# Autodesk Inventor assembly: 0005-00-03 Y axis
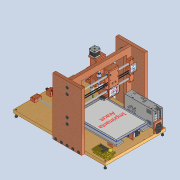
[picture p0: Inventor's stored thumbnail of the model, 180x180]
Saved by Autodesk Inventor 2020 (Build 240168000, 168)
## iProperties
Created: 2020-12-18
Part Number: 0005-00-03 Y axis
Document SubType Name: Assembly
Designer: Iulian Bors
Mass: 17144.8 g
Surface Area: 27601.7 cm^2
Volume: 16303.9 cm^3
Density: 1.05157 g/cm^3
Author: Iulian Bors
## iProperties of the stored document Part 1.ipt
Created: 2020-12-18
Part Number: Part 1
Material: Generic
Document SubType Name: Modeling
Designer: Iulian Bors
Density: 1 g/cm^3
Appearance: Default
Mass: 0.27605 g
Surface Area: 6.48852 cm^2
Volume: 0.27605 cm^3
Author: Iulian Bors
Revision Number: NONE
## iProperties of the stored document Part 2.ipt
Created: 2020-12-18
Part Number: Part 2
Material: Generic
Document SubType Name: Modeling
Designer: Iulian Bors
Density: 1 g/cm^3
Appearance: Default
Mass: 0.0253291 g
Surface Area: 2.0565 cm^2
Volume: 0.0253291 cm^3
Author: Iulian Bors
Revision Number: NONE
## iProperties of the stored document Needle.iam
Created: 2020-01-23
Part Number: Needle
Document SubType Name: Assembly
Designer: Iulian Bors
Mass: 0.301379 g
Surface Area: 8.54503 cm^2
Volume: 0.301379 cm^3
Density: 1 g/cm^3
Title: /vol/tmp/translate-4006329005178005204/5e293bbb2de6b7156cc2e2d4.step
## Documents named in this file (60)
- Z:\I.A.B\Proiecte\0005 I.A.B 3d 2.0 Imprimanta aracet\10 Mecanic\0005-00-03 Y axis.iam
- Z:\I.A.B\Proiecte\0005 I.A.B 3d 2.0 Imprimanta aracet\10 Mecanic\0005-10-001-Batiu.ipt
- Z:\I.A.B\Proiecte\0005 I.A.B 3d 2.0 Imprimanta aracet\20 Electric\0005-20-01 Assembly Arduino Mega RAMPS 1.4.iam
- Z:\I.A.B\Proiecte\0005 I.A.B 3d 2.0 Imprimanta aracet\10 Mecanic\Foaie A4.ipt
- Z:\I.A.B\Proiecte\0005 I.A.B 3d 2.0 Imprimanta aracet\10 Mecanic\Seringa\body 20ml_Défaut.ipt
- Z:\I.A.B\Proiecte\0005 I.A.B 3d 2.0 Imprimanta aracet\10 Mecanic\Seringa\Plunger Assembly_Défaut.iam
- **Z:\I.A.B\Proiecte\0005 I.A.B 3d 2.0 Imprimanta aracet\10 Mecanic\0005-00-03 Y axis.iam*LocalDocs*xAaaaqeaaAaaaaaaaAaaaq3zaLd*Needle.iam
- Z:\I.A.B\Proiecte\0005 I.A.B 3d 2.0 Imprimanta aracet\10 Mecanic\0005-10-003 Actionare seringa.ipt
- Z:\I.A.B\Proiecte\0005 I.A.B 3d 2.0 Imprimanta aracet\10 Mecanic\0005-10-004 Actionare 2 seringa.ipt
- Z:\I.A.B\Proiecte\0005 I.A.B 3d 2.0 Imprimanta aracet\10 Mecanic\0005-10-1004 Piulita.ipt
- Z:\I.A.B\Proiecte\0005 I.A.B 3d 2.0 Imprimanta aracet\10 Mecanic\0005-10-10-1003 LeadScrew 8mm x 2mmPitch.ipt
- Z:\I.A.B\Proiecte\0005 I.A.B 3d 2.0 Imprimanta aracet\10 Mecanic\0005-10-1005 ISO 1224-1 - 10 - 8 x 22 x 7.ipt
- Z:\I.A.B\Proiecte\0005 I.A.B 3d 2.0 Imprimanta aracet\10 Mecanic\0005-10-005.ipt
- Z:\I.A.B\Proiecte\0005 I.A.B 3d 2.0 Imprimanta aracet\10 Mecanic\0005-10-006 Capac rulment.ipt
- Z:\I.A.B\Proiecte\0005 I.A.B 3d 2.0 Imprimanta aracet\10 Mecanic\0005-10-1002  Hub.ipt
- Z:\I.A.B\Proiecte\0005 I.A.B 3d 2.0 Imprimanta aracet\10 Mecanic\0005-10-1001 NEMA17 - Motor de passo.ipt
- Z:\I.A.B\Proiecte\0005 I.A.B 3d 2.0 Imprimanta aracet\10 Mecanic\0005-10-007Suport nema.ipt
- Z:\I.A.B\Proiecte\0005 I.A.B 3d 2.0 Imprimanta aracet\10 Mecanic\0005-10-008.ipt
- Z:\I.A.B\Proiecte\0005 I.A.B 3d 2.0 Imprimanta aracet\10 Mecanic\0005-10-009.ipt
- Z:\I.A.B\Proiecte\0005 I.A.B 3d 2.0 Imprimanta aracet\10 Mecanic\0005-10-010.ipt
- Z:\I.A.B\Proiecte\0005 I.A.B 3d 2.0 Imprimanta aracet\10 Mecanic\0005-10-1006 Bara rectificata.ipt
- Z:\I.A.B\Proiecte\0005 I.A.B 3d 2.0 Imprimanta aracet\10 Mecanic\0005-10-011.ipt
- Z:\I.A.B\Proiecte\0005 I.A.B 3d 2.0 Imprimanta aracet\10 Mecanic\0005-10-012.ipt
- Z:\I.A.B\Proiecte\0005 I.A.B 3d 2.0 Imprimanta aracet\10 Mecanic\0005-10-1007 Bara rectificata.ipt
- Z:\I.A.B\Proiecte\0005 I.A.B 3d 2.0 Imprimanta aracet\10 Mecanic\0005-10-013 Bed.ipt
- Z:\I.A.B\Proiecte\0005 I.A.B 3d 2.0 Imprimanta aracet\10 Mecanic\0005-10-1008 Bara rectificata.ipt
- Z:\I.A.B\Proiecte\0005 I.A.B 3d 2.0 Imprimanta aracet\10 Mecanic\0005-10-014 Suport Bed.ipt
- Z:\I.A.B\Proiecte\0005 I.A.B 3d 2.0 Imprimanta aracet\10 Mecanic\0005-10-1009 LM10uu.ipt
- Z:\I.A.B\Proiecte\0005 I.A.B 3d 2.0 Imprimanta aracet\10 Mecanic\0005-10-002 Suport1 Seringa.ipt
- Z:\I.A.B\Proiecte\0005 I.A.B 3d 2.0 Imprimanta aracet\10 Mecanic\0005-10-016.ipt
- Z:\I.A.B\Proiecte\0005 I.A.B 3d 2.0 Imprimanta aracet\10 Mecanic\0005-10-015 suport tija.ipt
- Z:\I.A.B\Proiecte\0005 I.A.B 3d 2.0 Imprimanta aracet\10 Mecanic\0005-10-017 Batiu 2.ipt
- Z:\I.A.B\Proiecte\0005 I.A.B 3d 2.0 Imprimanta aracet\10 Mecanic\0005-10-1010 GT2 Timing Pulley 20 Tooth.ipt
- Z:\I.A.B\Proiecte\0005 I.A.B 3d 2.0 Imprimanta aracet\10 Mecanic\0005-10-1011 16T W6 B3 Without T_Shrinkwrap_1.ipt
- Z:\I.A.B\Proiecte\0005 I.A.B 3d 2.0 Imprimanta aracet\10 Mecanic\Surub M4 saiba piulita.iam
- Z:\I.A.B\Proiecte\0005 I.A.B 3d 2.0 Imprimanta aracet\10 Mecanic\0005-10-018 intinzator x.ipt
- Z:\I.A.B\Proiecte\0005 I.A.B 3d 2.0 Imprimanta aracet\10 Mecanic\0005-10-1015 curea x.ipt
- Z:\I.A.B\Proiecte\0005 I.A.B 3d 2.0 Imprimanta aracet\10 Mecanic\0005-10-019 intinzator y.ipt
- Z:\I.A.B\Proiecte\0005 I.A.B 3d 2.0 Imprimanta aracet\10 Mecanic\0005-10-1016 curea Y.ipt
- Z:\I.A.B\Proiecte\0005 I.A.B 3d 2.0 Imprimanta aracet\20 Electric\0005-20-1003 Switch.ipt
- Z:\I.A.B\Proiecte\0005 I.A.B 3d 2.0 Imprimanta aracet\10 Mecanic\0005-10-021 suport senzor z.ipt
- Z:\I.A.B\Proiecte\0005 I.A.B 3d 2.0 Imprimanta aracet\10 Mecanic\0005-10-020 suport motor y.ipt
- Z:\I.A.B\Proiecte\0005 I.A.B 3d 2.0 Imprimanta aracet\10 Mecanic\0005-10-023 Suport motor x.ipt
- Z:\I.A.B\Proiecte\0005 I.A.B 3d 2.0 Imprimanta aracet\10 Mecanic\0005-10-024.ipt
- Z:\I.A.B\Proiecte\0005 I.A.B 3d 2.0 Imprimanta aracet\10 Mecanic\0005-10-1000 LM8.ipt
- Z:\I.A.B\Proiecte\0005 I.A.B 3d 2.0 Imprimanta aracet\10 Mecanic\0005-10-1018 tija 8.ipt
- Z:\I.A.B\Proiecte\0005 I.A.B 3d 2.0 Imprimanta aracet\10 Mecanic\Surub M3 40 mm.iam
- Z:\I.A.B\Proiecte\0005 I.A.B 3d 2.0 Imprimanta aracet\10 Mecanic\0005-10-025 Activator senzor Y.ipt
- Z:\I.A.B\Proiecte\0005 I.A.B 3d 2.0 Imprimanta aracet\10 Mecanic\0005-10-1022 tiping screw.ipt
- Z:\I.A.B\Proiecte\0005 I.A.B 3d 2.0 Imprimanta aracet\10 Mecanic\0005-10-1023 ISO 4018 - M8 x 40.ipt
- Z:\I.A.B\Proiecte\0005 I.A.B 3d 2.0 Imprimanta aracet\10 Mecanic\0005-10-026 Suport DC in.ipt
- Z:\I.A.B\Proiecte\0005 I.A.B 3d 2.0 Imprimanta aracet\20 Electric\00005-20-1004 PowerSupplyLedMax500.ipt
- Z:\I.A.B\Proiecte\0005 I.A.B 3d 2.0 Imprimanta aracet\20 Electric\005-20-1004.ipt
- Z:\I.A.B\Proiecte\0005 I.A.B 3d 2.0 Imprimanta aracet\10 Mecanic\0005-10-027 suport nema Z.ipt
- Z:\I.A.B\Proiecte\0005 I.A.B 3d 2.0 Imprimanta aracet\10 Mecanic\0005-10-1025 ISO 4762 - M3 x 16ISO.ipt
- Z:\I.A.B\Proiecte\0005 I.A.B 3d 2.0 Imprimanta aracet\10 Mecanic\0005-10-1020 ISO 7089 - 3 - 140 HV(1).ipt
- **Z:\I.A.B\Proiecte\0005 I.A.B 3d 2.0 Imprimanta aracet\0005-00-00 Ansamblu_General.iam*LocalDocs*xAaaaaecaAaaaaaaaAaaaqfy1Od*Part 1.ipt
- **Z:\I.A.B\Proiecte\0005 I.A.B 3d 2.0 Imprimanta aracet\0005-00-00 Ansamblu_General.iam*LocalDocs*xAaaaa4baAaaaaaaaAaaaq4bsZa*Part 2.ipt
- **Z:\I.A.B\Proiecte\0005 I.A.B 3d 2.0 Imprimanta aracet\0005-00-00 Ansamblu_General.iam*LocalDocs*xAaaaqeaaAaaaaaaaAaaaq3zaLd*Needle.iam
- Z:\I.A.B\Proiecte\0005 I.A.B 3d 2.0 Imprimanta aracet\10 Mecanic\Seringa\21-gauge-needle-1.snapshot.2\Needle.step
## Components (116 placed, 54 different names)
1. 0005-10-001-Batiu.ipt:1 — Mate:3, Angle:1, Mate:43, Angle:7, Angle:8, Angle:10, Mate:62, Flush:36, Mate:64, Flush:38, Mate:109, Mate:90, Mate:91, Mate:92, Mate:93, Mate:101, Mate:108, Flush:60, Mate:116, Insert:32, Insert:33, Mate:127, Mate:131, Mate:143, Mate:147, Flush:73, Insert:41, Insert:42
2. 0005-20-01 Assembly Arduino Mega RAMPS 1.4.iam:2 [sub-assembly] — Mate:147, Flush:73
3. Foaie A4.ipt:3 — Mate:3, Angle:1, Flush:29, Flush:30, Mate:47
4. Needle.iam:4 [sub-assembly] — Insert:14
5. 0005-10-10-1003 LeadScrew 8mm x 2mmPitch.ipt:5 — Insert:2, Insert:4, Mate:61, Mate:118
6. 0005-10-1005 ISO 1224-1 - 10 - 8 x 22 x 7.ipt:6 — Insert:2, Mate:15, Insert:3
7. 0005-10-005.ipt:7 — Mate:15, Mate:16, Flush:4, Flush:5, Mate:17, Flush:6, Flush:7, Mate:18, Mate:50, Mate:51, Angle:9, Mate:59, Mate:61, Flush:35, Mate:137, Mate:138
8. 0005-10-006 Capac rulment.ipt:8 — Insert:3
9. 0005-10-1002  Hub.ipt:9 — Insert:4, Insert:5
10. 0005-10-1001 NEMA17 - Motor de passo.ipt:10 — Insert:5
11. 0005-10-008.ipt:11 — Mate:16, Flush:4, Flush:5, Flush:11, Mate:21, Mate:22, Angle:11
12. 0005-10-008.ipt:12 — Mate:17, Flush:6, Flush:7, Mate:119, Flush:64
13. 0005-10-016.ipt:13 — Mate:18, Mate:19, Mate:20, Mate:28, Flush:12, Flush:18, Flush:35, Flush:63
14. 0005-10-009.ipt:14 — Mate:19, Flush:11, Flush:18, Flush:63, Flush:65
15. 0005-10-010.ipt:15 — Mate:20, Mate:21, Mate:22, Insert:7, Mate:35, Mate:37, Mate:103, Insert:26, Insert:27
16. 0005-10-1004 Piulita.ipt:16 — Mate:35, Mate:36
17. 0005-10-1009 LM10uu.ipt:17 — Insert:7, Mate:26, Flush:57
18. 0005-10-1006 Bara rectificata.ipt:18 — Mate:26, Flush:27
19. 0005-10-1006 Bara rectificata.ipt:19 — Flush:14, Mate:103, Mate:104
20. 0005-10-011.ipt:20 — Mate:28, Flush:12, Flush:14, Mate:32, Angle:5, Flush:27, Mate:98, Flush:53, Insert:36, Flush:69, Flush:70, Mate:151, Flush:74
21. 0005-10-10-1003 LeadScrew 8mm x 2mmPitch.ipt:21 — Mate:33, Mate:36, Mate:37, Insert:37, Insert:38
22. 0005-10-1002  Hub.ipt:22 — Mate:33
23. 0005-10-1001 NEMA17 - Motor de passo.ipt:23 — Mate:32, Angle:5, Insert:37
24. 0005-10-011.ipt:24 — Insert:40, Mate:142, Flush:71, Flush:72
25. 0005-10-012.ipt:25 — Flush:22, Flush:25, Flush:26, Mate:40, Mate:56, Mate:57, Mate:71, Mate:72, Flush:44, Mate:142, Mate:151
26. 0005-10-006 Capac rulment.ipt:26 — Insert:39
27. 0005-10-1005 ISO 1224-1 - 10 - 8 x 22 x 7.ipt:27 — Insert:38, Insert:39
28. 0005-10-1009 LM10uu.ipt:28 — Flush:22, Mate:41, Mate:49, Mate:56, Mate:57
29. 0005-10-012.ipt:29 — Flush:25, Flush:34, Flush:26, Mate:40, Mate:43, Insert:18, Insert:19, Insert:20, Flush:69, Flush:70, Flush:71, Flush:72
30. 0005-10-1007 Bara rectificata.ipt:30 — Mate:41, Angle:13, Mate:68, Mate:70, Flush:43
31. 0005-10-014 Suport Bed.ipt:31 — Flush:28, Tangent:11, Tangent:12, Angle:7, Angle:8, Flush:29, Flush:30, Mate:46, Flush:32, Flush:33, Mate:48, Mate:125, Flush:67
32. 0005-10-013 Bed.ipt:36 — Mate:47, Flush:32, Flush:33, Mate:48
33. 0005-10-1009 LM10uu.ipt:37 — Mate:49, Flush:34, Flush:45
34. 0005-10-1004 Piulita.ipt:38 — Insert:13
35. body 20ml_Défaut.ipt:39 — Mate:50, Mate:51, Angle:9, Mate:52, Insert:14
36. 0005-10-017 Batiu 2.ipt:50 — Mate:109, Mate:66, Mate:67, Flush:41, Mate:69, Flush:42, Mate:75, Mate:77, Flush:46, Flush:47, Angle:15, Mate:111, Mate:112, Mate:113, Mate:114, Mate:115, Flush:62, Mate:123, Mate:144, Mate:145, Mate:148, Mate:150
37. Plunger Assembly_Défaut.iam:40 [sub-assembly] — Mate:52, Angle:10, Mate:53
38. 0005-10-003 Actionare seringa.ipt:41 — Insert:13, Mate:53, Angle:11, Mate:117, Mate:118, Insert:22, Mate:121, Mate:122
39. 0005-10-004 Actionare 2 seringa.ipt:42 — Insert:22, Mate:122
40. 0005-10-002 Suport1 Seringa.ipt:43 — Mate:59, Mate:137, Mate:138
41. 0005-10-015 suport tija.ipt:51 — Mate:67, Mate:68, Flush:41, Flush:43
42. 0005-10-015 suport tija.ipt:52 — Mate:69, Mate:70, Flush:42, Mate:82, Insert:24
43. 0005-10-1009 LM10uu.ipt:53 — Mate:71, Mate:72, Flush:44, Mate:73, Mate:74
44. 0005-10-1009 LM10uu.ipt:54 — Flush:45, Mate:73
45. 0005-10-1007 Bara rectificata.ipt:55 — Mate:74, Mate:76, Mate:78, Flush:48
46. 0005-10-015 suport tija.ipt:56 — Mate:75, Mate:76, Flush:47, Flush:48
47. 0005-10-015 suport tija.ipt:57 — Mate:77, Mate:78, Flush:46
48. 0005-10-1001 NEMA17 - Motor de passo.ipt:58 — Mate:144, Mate:145, Mate:146
49. 0005-10-1010 GT2 Timing Pulley 20 Tooth.ipt:59 — Flush:49, Mate:83, Mate:84, Mate:110, Mate:146
50. 0005-10-1011 16T W6 B3 Without T_Shrinkwrap_1.ipt:60 — Flush:49, Mate:80, Mate:81, Mate:83
51. 0005-10-018 intinzator x.ipt:61 — Mate:80, Mate:81, Mate:82, Insert:16, Insert:17, Mate:111
52. 0005-10-023 Suport motor x.ipt:62 — Mate:112, Mate:113
53. Surub M4 saiba piulita.iam:63 [sub-assembly] — Insert:16
54. Surub M4 saiba piulita.iam:64 [sub-assembly] — Insert:17
55. Surub M4 saiba piulita.iam:65 [sub-assembly] — Insert:18
56. Surub M4 saiba piulita.iam:66 [sub-assembly] — Insert:20
57. Surub M4 saiba piulita.iam:67 [sub-assembly] — Insert:19
58. 0005-10-1015 curea x.ipt:68 — Angle:15, Mate:84, Mate:110
59. 0005-10-1001 NEMA17 - Motor de passo.ipt:69 — Mate:90, Mate:102, Flush:55, Flush:58
60. 0005-10-1010 GT2 Timing Pulley 20 Tooth.ipt:70 — Mate:94, Mate:95, Flush:51
61. 0005-10-1011 16T W6 B3 Without T_Shrinkwrap_1.ipt:71 — Flush:51
62. 0005-10-019 intinzator y.ipt:72 — Mate:91, Mate:92, Mate:93, Angle:17
63. 0005-10-1016 curea Y.ipt:73 — Mate:94, Mate:95, Angle:17
64. 0005-20-1003 Switch.ipt:74 — Mate:123
65. 0005-10-021 suport senzor z.ipt:75 — Mate:98, Flush:53, Mate:99, Flush:54, Flush:74
66. 0005-20-1003 Switch.ipt:76 — Mate:99, Flush:54
67. 0005-20-1003 Switch.ipt:77 — Mate:100
68. 0005-10-020 suport motor y.ipt:78 — Mate:101, Mate:102, Flush:55
69. 0005-10-1009 LM10uu.ipt:79 — Mate:104, Flush:57
70. Inlet Module Plug Fuse Switch Male Power Socket 10A 250V 3 Pin IEC320 C14.ipt:82 — Mate:108, Mate:129, Mate:131, Mate:132
71. 0005-10-024.ipt:83 — Flush:60, Mate:114, Mate:115, Flush:61, Insert:28, Mate:126
72. 0005-10-024.ipt:84 — Mate:116, Flush:61, Flush:62, Insert:29, Insert:30, Mate:149
73. 0005-10-1000 LM8.ipt:85 — Mate:117, Mate:120
74. 0005-10-007Suport nema.ipt:86 — Mate:119, Flush:64, Flush:65, Flush:66
75. 0005-10-1018 tija 8.ipt:87 — Mate:120, Mate:121, Flush:66
76. Surub M4 saiba piulita.iam:88 [sub-assembly] — Insert:24
77. Surub M3 40 mm.iam:89 [sub-assembly] — Insert:40
78. 0005-10-025 Activator senzor Y.ipt:90 — Mate:125, Flush:67, Flush:68
79. 0005-10-1009 LM10uu.ipt:91 — Insert:27
80. 0005-10-1009 LM10uu.ipt:92 — Insert:26
81. 0005-10-1023 ISO 4018 - M8 x 40.ipt:121 — Insert:41
82. 0005-10-1023 ISO 4018 - M8 x 40.ipt:122 — Insert:32
83. 0005-10-1023 ISO 4018 - M8 x 40.ipt:123 — Insert:33
84. 0005-10-1023 ISO 4018 - M8 x 40.ipt:124 — Insert:42
85. 0005-10-026 Suport DC in.ipt:125 — Mate:127, Mate:129, Mate:132
86. 00005-20-1004 PowerSupplyLedMax500.ipt:126 — Mate:143, Mate:148, Mate:149
87. ISO 4762 M3 x 16:1 — Insert:35, Insert:36
88. ISO 7089 3:1 — Insert:35
89. 0005-10-1009 LM10uu.ipt:32 — Flush:28, Tangent:11, Tangent:12
90. 0005-10-1009 LM10uu.ipt:33 — Mate:44, Mate:63
91. 0005-10-1009 LM10uu.ipt:34 — Flush:68
92. 0005-10-1009 LM10uu.ipt:35 — Mate:65
93. 0005-10-015 suport tija.ipt:44 — Mate:62, Mate:63, Flush:36, Flush:37
94. 0005-10-015 suport tija.ipt:45 — Mate:64, Mate:65, Flush:38
95. 0005-10-1008 Bara rectificata.ipt:46 — Mate:44, Flush:37
96. 0005-10-015 suport tija.ipt:47
97. 0005-10-015 suport tija.ipt:48 — Mate:100
98. 0005-10-1008 Bara rectificata.ipt:49
99. 0005-10-1022 tiping screw.ipt:93 — Insert:28
100. 0005-10-1022 tiping screw.ipt:94
101. 0005-10-1022 tiping screw.ipt:95
102. 0005-10-1022 tiping screw.ipt:96
103. 0005-10-1022 tiping screw.ipt:102 — Mate:126
104. 0005-10-1022 tiping screw.ipt:103
105. 0005-10-1022 tiping screw.ipt:104
106. 0005-10-1022 tiping screw.ipt:105
107. 0005-10-1022 tiping screw.ipt:106
108. 0005-10-1022 tiping screw.ipt:107 — Insert:29
109. 0005-10-1022 tiping screw.ipt:108
110. 0005-10-1022 tiping screw.ipt:109
111. 0005-10-1022 tiping screw.ipt:110
112. 0005-10-1022 tiping screw.ipt:116 — Insert:30
113. 0005-10-1022 tiping screw.ipt:117
114. 0005-10-1022 tiping screw.ipt:118
115. 0005-10-1022 tiping screw.ipt:119
116. 0005-10-1022 tiping screw.ipt:120
## Component patterns: (4 elements, first: 0005-10-1009 LM10uu.ipt:32), (2 elements, first: 0005-10-015 suport tija.ipt:44 + 0005-10-015 suport tija.ipt:45 + 0005-10-1008 Bara rectificata.ipt:46), (4 elements, first: 0005-10-1022 tiping screw.ipt:93), (5 elements, first: 0005-10-1022 tiping screw.ipt:102), (4 elements, first: 0005-10-1022 tiping screw.ipt:107), (5 elements, first: 0005-10-1022 tiping screw.ipt:116)
## Relationships (198: Mate 103, Flush 52, Insert 31, Angle 10, Tangent 2)
- Mate:3 (53 mm): 0005-10-001-Batiu.ipt:1 ↔ Foaie A4.ipt:3
- Angle:1 (0 deg): 0005-10-001-Batiu.ipt:1 ↔ Foaie A4.ipt:3
- Insert:2: 0005-10-10-1003 LeadScrew 8mm x 2mmPitch.ipt:5 ↔ 0005-10-1005 ISO 1224-1 - 10 - 8 x 22 x 7.ipt:6
- Mate:15: 0005-10-1005 ISO 1224-1 - 10 - 8 x 22 x 7.ipt:6 ↔ 0005-10-005.ipt:7
- Insert:3: 0005-10-1005 ISO 1224-1 - 10 - 8 x 22 x 7.ipt:6 ↔ 0005-10-006 Capac rulment.ipt:8
- Insert:4: 0005-10-10-1003 LeadScrew 8mm x 2mmPitch.ipt:5 ↔ 0005-10-1002  Hub.ipt:9
- Insert:5 (5 mm): 0005-10-1002  Hub.ipt:9 ↔ 0005-10-1001 NEMA17 - Motor de passo.ipt:10
- Mate:16: 0005-10-005.ipt:7 ↔ 0005-10-008.ipt:11
- Flush:4: 0005-10-005.ipt:7 ↔ 0005-10-008.ipt:11
- Flush:5: 0005-10-005.ipt:7 ↔ 0005-10-008.ipt:11
- Mate:17: 0005-10-005.ipt:7 ↔ 0005-10-008.ipt:12
- Flush:6: 0005-10-005.ipt:7 ↔ 0005-10-008.ipt:12
- Flush:7: 0005-10-005.ipt:7 ↔ 0005-10-008.ipt:12
- Mate:18: 0005-10-005.ipt:7 ↔ 0005-10-016.ipt:13
- Mate:19 (8 mm): 0005-10-016.ipt:13 ↔ 0005-10-009.ipt:14
- Flush:11: 0005-10-008.ipt:11 ↔ 0005-10-009.ipt:14
- Mate:20: 0005-10-016.ipt:13 ↔ 0005-10-010.ipt:15
- Mate:21: 0005-10-008.ipt:11 ↔ 0005-10-010.ipt:15
- Mate:22: 0005-10-008.ipt:11 ↔ 0005-10-010.ipt:15
- Insert:7: 0005-10-010.ipt:15 ↔ 0005-10-1009 LM10uu.ipt:17
- Mate:26: 0005-10-1009 LM10uu.ipt:17 ↔ 0005-10-1006 Bara rectificata.ipt:18
- Mate:28 (3 mm): 0005-10-016.ipt:13 ↔ 0005-10-011.ipt:20
- Flush:12: 0005-10-016.ipt:13 ↔ 0005-10-011.ipt:20
- Flush:14: 0005-10-1006 Bara rectificata.ipt:19 ↔ 0005-10-011.ipt:20
- [Insert] (5 mm): 0005-10-1002  Hub.ipt:22 ↔ 0005-10-1001 NEMA17 - Motor de passo.ipt:23
- Mate:32: 0005-10-011.ipt:20 ↔ 0005-10-1001 NEMA17 - Motor de passo.ipt:23
- Mate:33: 0005-10-10-1003 LeadScrew 8mm x 2mmPitch.ipt:21 ↔ 0005-10-1002  Hub.ipt:22
- Angle:5 (0 deg): 0005-10-011.ipt:20 ↔ 0005-10-1001 NEMA17 - Motor de passo.ipt:23
- Mate:35: 0005-10-010.ipt:15 ↔ 0005-10-1004 Piulita.ipt:16
- Mate:36: 0005-10-1004 Piulita.ipt:16 ↔ 0005-10-10-1003 LeadScrew 8mm x 2mmPitch.ipt:21
- Mate:37: 0005-10-010.ipt:15 ↔ 0005-10-10-1003 LeadScrew 8mm x 2mmPitch.ipt:21
- Flush:18: 0005-10-016.ipt:13 ↔ 0005-10-009.ipt:14
- Flush:22: 0005-10-012.ipt:25 ↔ 0005-10-1009 LM10uu.ipt:28
- Flush:25: 0005-10-012.ipt:25 ↔ 0005-10-012.ipt:29
- Flush:34: 0005-10-012.ipt:29 ↔ 0005-10-1009 LM10uu.ipt:37
- Flush:26: 0005-10-012.ipt:25 ↔ 0005-10-012.ipt:29
- Mate:40 (19 mm): 0005-10-012.ipt:25 ↔ 0005-10-012.ipt:29
- Flush:27: 0005-10-1006 Bara rectificata.ipt:18 ↔ 0005-10-011.ipt:20
- Mate:41: 0005-10-1009 LM10uu.ipt:28 ↔ 0005-10-1007 Bara rectificata.ipt:30
- Mate:43 (173.806 mm): 0005-10-001-Batiu.ipt:1 ↔ 0005-10-012.ipt:29
- Flush:28 (75 mm): 0005-10-014 Suport Bed.ipt:31 ↔ 0005-10-1009 LM10uu.ipt:32
- Tangent:11: 0005-10-014 Suport Bed.ipt:31 ↔ 0005-10-1009 LM10uu.ipt:32
- Tangent:12 (-20 mm): 0005-10-014 Suport Bed.ipt:31 ↔ 0005-10-1009 LM10uu.ipt:32
- Angle:7 (0 deg): 0005-10-001-Batiu.ipt:1 ↔ 0005-10-014 Suport Bed.ipt:31
- Angle:8 (0 deg): 0005-10-001-Batiu.ipt:1 ↔ 0005-10-014 Suport Bed.ipt:31
- Mate:44: 0005-10-1009 LM10uu.ipt:33 ↔ 0005-10-1008 Bara rectificata.ipt:46
- Flush:29 (10 mm): Foaie A4.ipt:3 ↔ 0005-10-014 Suport Bed.ipt:31
- Flush:30 (12.5 mm): Foaie A4.ipt:3 ↔ 0005-10-014 Suport Bed.ipt:31
- Mate:46 (18 mm): 0005-10-014 Suport Bed.ipt:31
- Mate:47: Foaie A4.ipt:3 ↔ 0005-10-013 Bed.ipt:36
- Flush:32: 0005-10-014 Suport Bed.ipt:31 ↔ 0005-10-013 Bed.ipt:36
- Flush:33: 0005-10-014 Suport Bed.ipt:31 ↔ 0005-10-013 Bed.ipt:36
- Mate:48 (20 mm): 0005-10-014 Suport Bed.ipt:31 ↔ 0005-10-013 Bed.ipt:36
- Mate:49: 0005-10-1009 LM10uu.ipt:28 ↔ 0005-10-1009 LM10uu.ipt:37
- Mate:50: 0005-10-005.ipt:7 ↔ body 20ml_Défaut.ipt:39
- Mate:51: 0005-10-005.ipt:7 ↔ body 20ml_Défaut.ipt:39
- Angle:9 (0 deg): 0005-10-005.ipt:7 ↔ body 20ml_Défaut.ipt:39
- Mate:52: body 20ml_Défaut.ipt:39 ↔ Plunger Assembly_Défaut.iam:40
- Angle:10 (0 deg): 0005-10-001-Batiu.ipt:1 ↔ Plunger Assembly_Défaut.iam:40
- Insert:13: 0005-10-1004 Piulita.ipt:38 ↔ 0005-10-003 Actionare seringa.ipt:41
- Mate:53: Plunger Assembly_Défaut.iam:40 ↔ 0005-10-003 Actionare seringa.ipt:41
- Insert:14 (-5 mm): Needle.iam:4 ↔ body 20ml_Défaut.ipt:39
- Mate:56 (9.5 mm): 0005-10-012.ipt:25 ↔ 0005-10-1009 LM10uu.ipt:28
- Mate:57 (-30 mm): 0005-10-012.ipt:25 ↔ 0005-10-1009 LM10uu.ipt:28
- Angle:11 (0 deg): 0005-10-008.ipt:11 ↔ 0005-10-003 Actionare seringa.ipt:41
- Mate:59: 0005-10-005.ipt:7 ↔ 0005-10-002 Suport1 Seringa.ipt:43
- Mate:61: 0005-10-10-1003 LeadScrew 8mm x 2mmPitch.ipt:5 ↔ 0005-10-005.ipt:7
- Flush:35: 0005-10-005.ipt:7 ↔ 0005-10-016.ipt:13
- Mate:62: 0005-10-001-Batiu.ipt:1 ↔ 0005-10-015 suport tija.ipt:44
- Mate:63: 0005-10-1009 LM10uu.ipt:33 ↔ 0005-10-015 suport tija.ipt:44
- Flush:36 (5.193 mm): 0005-10-001-Batiu.ipt:1 ↔ 0005-10-015 suport tija.ipt:44
- Mate:64: 0005-10-001-Batiu.ipt:1 ↔ 0005-10-015 suport tija.ipt:45
- Flush:37: 0005-10-015 suport tija.ipt:44 ↔ 0005-10-1008 Bara rectificata.ipt:46
- Mate:65: 0005-10-1009 LM10uu.ipt:35 ↔ 0005-10-015 suport tija.ipt:45
- Flush:38 (66.773 mm): 0005-10-001-Batiu.ipt:1 ↔ 0005-10-015 suport tija.ipt:45
- Mate:109: 0005-10-001-Batiu.ipt:1 ↔ 0005-10-017 Batiu 2.ipt:50
- Mate:66: 0005-10-017 Batiu 2.ipt:50
- Angle:13 (0 deg): 0005-10-1007 Bara rectificata.ipt:30
- Mate:67: 0005-10-017 Batiu 2.ipt:50 ↔ 0005-10-015 suport tija.ipt:51
- Mate:68: 0005-10-1007 Bara rectificata.ipt:30 ↔ 0005-10-015 suport tija.ipt:51
- Flush:41: 0005-10-017 Batiu 2.ipt:50 ↔ 0005-10-015 suport tija.ipt:51
- Mate:69: 0005-10-017 Batiu 2.ipt:50 ↔ 0005-10-015 suport tija.ipt:52
- Mate:70: 0005-10-1007 Bara rectificata.ipt:30 ↔ 0005-10-015 suport tija.ipt:52
- Flush:42: 0005-10-017 Batiu 2.ipt:50 ↔ 0005-10-015 suport tija.ipt:52
- Flush:43: 0005-10-1007 Bara rectificata.ipt:30 ↔ 0005-10-015 suport tija.ipt:51
- Mate:71: 0005-10-012.ipt:25 ↔ 0005-10-1009 LM10uu.ipt:53
- Mate:72 (9.5 mm): 0005-10-012.ipt:25 ↔ 0005-10-1009 LM10uu.ipt:53
- Flush:44 (30 mm): 0005-10-012.ipt:25 ↔ 0005-10-1009 LM10uu.ipt:53
- Flush:45: 0005-10-1009 LM10uu.ipt:37 ↔ 0005-10-1009 LM10uu.ipt:54
- Mate:73: 0005-10-1009 LM10uu.ipt:53 ↔ 0005-10-1009 LM10uu.ipt:54
- Mate:74: 0005-10-1009 LM10uu.ipt:53 ↔ 0005-10-1007 Bara rectificata.ipt:55
- Mate:75: 0005-10-017 Batiu 2.ipt:50 ↔ 0005-10-015 suport tija.ipt:56
- Mate:76: 0005-10-1007 Bara rectificata.ipt:55 ↔ 0005-10-015 suport tija.ipt:56
- Mate:77: 0005-10-017 Batiu 2.ipt:50 ↔ 0005-10-015 suport tija.ipt:57
- Mate:78: 0005-10-1007 Bara rectificata.ipt:55 ↔ 0005-10-015 suport tija.ipt:57
- Flush:46: 0005-10-017 Batiu 2.ipt:50 ↔ 0005-10-015 suport tija.ipt:57
- Flush:47: 0005-10-017 Batiu 2.ipt:50 ↔ 0005-10-015 suport tija.ipt:56
- Flush:48: 0005-10-1007 Bara rectificata.ipt:55 ↔ 0005-10-015 suport tija.ipt:56
- Flush:49: 0005-10-1010 GT2 Timing Pulley 20 Tooth.ipt:59 ↔ 0005-10-1011 16T W6 B3 Without T_Shrinkwrap_1.ipt:60
- Mate:80: 0005-10-1011 16T W6 B3 Without T_Shrinkwrap_1.ipt:60 ↔ 0005-10-018 intinzator x.ipt:61
- Mate:81 (1 mm): 0005-10-1011 16T W6 B3 Without T_Shrinkwrap_1.ipt:60 ↔ 0005-10-018 intinzator x.ipt:61
- Mate:82 (5 mm): 0005-10-015 suport tija.ipt:52 ↔ 0005-10-018 intinzator x.ipt:61
- Mate:83: 0005-10-1010 GT2 Timing Pulley 20 Tooth.ipt:59 ↔ 0005-10-1011 16T W6 B3 Without T_Shrinkwrap_1.ipt:60
- Insert:16: 0005-10-018 intinzator x.ipt:61 ↔ Surub M4 saiba piulita.iam:63
- Insert:17: 0005-10-018 intinzator x.ipt:61 ↔ Surub M4 saiba piulita.iam:64
- Insert:18: 0005-10-012.ipt:29 ↔ Surub M4 saiba piulita.iam:65
- Insert:19: 0005-10-012.ipt:29 ↔ Surub M4 saiba piulita.iam:67
- Insert:20: 0005-10-012.ipt:29 ↔ Surub M4 saiba piulita.iam:66
- Angle:15 (0 deg): 0005-10-017 Batiu 2.ipt:50 ↔ 0005-10-1015 curea x.ipt:68
- Mate:84: 0005-10-1010 GT2 Timing Pulley 20 Tooth.ipt:59 ↔ 0005-10-1015 curea x.ipt:68
- [Insert] (-13 mm): 0005-10-1001 NEMA17 - Motor de passo.ipt:69 ↔ 0005-10-1010 GT2 Timing Pulley 20 Tooth.ipt:70
- [Mate]: 0005-10-1011 16T W6 B3 Without T_Shrinkwrap_1.ipt:71 ↔ 0005-10-019 intinzator y.ipt:72
- [Mate] (1 mm): 0005-10-1011 16T W6 B3 Without T_Shrinkwrap_1.ipt:71 ↔ 0005-10-019 intinzator y.ipt:72
- Mate:90: 0005-10-001-Batiu.ipt:1 ↔ 0005-10-1001 NEMA17 - Motor de passo.ipt:69
- Mate:91: 0005-10-001-Batiu.ipt:1 ↔ 0005-10-019 intinzator y.ipt:72
- Mate:92: 0005-10-001-Batiu.ipt:1 ↔ 0005-10-019 intinzator y.ipt:72
- Mate:93: 0005-10-001-Batiu.ipt:1 ↔ 0005-10-019 intinzator y.ipt:72
- Mate:94: 0005-10-1010 GT2 Timing Pulley 20 Tooth.ipt:70 ↔ 0005-10-1016 curea Y.ipt:73
- Mate:95: 0005-10-1010 GT2 Timing Pulley 20 Tooth.ipt:70 ↔ 0005-10-1016 curea Y.ipt:73
- Flush:51: 0005-10-1010 GT2 Timing Pulley 20 Tooth.ipt:70 ↔ 0005-10-1011 16T W6 B3 Without T_Shrinkwrap_1.ipt:71
- Angle:17 (0 deg): 0005-10-019 intinzator y.ipt:72 ↔ 0005-10-1016 curea Y.ipt:73
- Mate:98: 0005-10-011.ipt:20 ↔ 0005-10-021 suport senzor z.ipt:75
- Flush:53 (-15 mm): 0005-10-011.ipt:20 ↔ 0005-10-021 suport senzor z.ipt:75
- Mate:99: 0005-10-021 suport senzor z.ipt:75 ↔ 0005-20-1003 Switch.ipt:76
- Flush:54: 0005-10-021 suport senzor z.ipt:75 ↔ 0005-20-1003 Switch.ipt:76
- Mate:100: 0005-20-1003 Switch.ipt:77 ↔ 0005-10-015 suport tija.ipt:48
- Mate:101: 0005-10-001-Batiu.ipt:1 ↔ 0005-10-020 suport motor y.ipt:78
- Mate:102: 0005-10-1001 NEMA17 - Motor de passo.ipt:69 ↔ 0005-10-020 suport motor y.ipt:78
- Flush:55: 0005-10-1001 NEMA17 - Motor de passo.ipt:69 ↔ 0005-10-020 suport motor y.ipt:78
- Mate:103: 0005-10-010.ipt:15 ↔ 0005-10-1006 Bara rectificata.ipt:19
- Mate:104: 0005-10-1006 Bara rectificata.ipt:19 ↔ 0005-10-1009 LM10uu.ipt:79
- Flush:57: 0005-10-1009 LM10uu.ipt:17 ↔ 0005-10-1009 LM10uu.ipt:79
- Flush:58 (-322.09 mm): 0005-10-1001 NEMA17 - Motor de passo.ipt:69
- Mate:108: 0005-10-001-Batiu.ipt:1 ↔ Inlet Module Plug Fuse Switch Male Power Socket 10A 250V 3 Pin IEC320 C14.ipt:82
- Mate:110: 0005-10-1010 GT2 Timing Pulley 20 Tooth.ipt:59 ↔ 0005-10-1015 curea x.ipt:68
- Mate:111: 0005-10-017 Batiu 2.ipt:50 ↔ 0005-10-018 intinzator x.ipt:61
- Mate:112: 0005-10-017 Batiu 2.ipt:50 ↔ 0005-10-023 Suport motor x.ipt:62
- Mate:113 (-10 mm): 0005-10-017 Batiu 2.ipt:50 ↔ 0005-10-023 Suport motor x.ipt:62
- Flush:60: 0005-10-001-Batiu.ipt:1 ↔ 0005-10-024.ipt:83
- Mate:114: 0005-10-017 Batiu 2.ipt:50 ↔ 0005-10-024.ipt:83
- Mate:115: 0005-10-017 Batiu 2.ipt:50 ↔ 0005-10-024.ipt:83
- Mate:116: 0005-10-001-Batiu.ipt:1 ↔ 0005-10-024.ipt:84
- Flush:61: 0005-10-024.ipt:83 ↔ 0005-10-024.ipt:84
- Flush:62: 0005-10-017 Batiu 2.ipt:50 ↔ 0005-10-024.ipt:84
- Mate:117 (-10 mm): 0005-10-003 Actionare seringa.ipt:41 ↔ 0005-10-1000 LM8.ipt:85
- Mate:118: 0005-10-10-1003 LeadScrew 8mm x 2mmPitch.ipt:5 ↔ 0005-10-003 Actionare seringa.ipt:41
- Flush:63: 0005-10-016.ipt:13 ↔ 0005-10-009.ipt:14
- Insert:22 (1 mm): 0005-10-003 Actionare seringa.ipt:41 ↔ 0005-10-004 Actionare 2 seringa.ipt:42
- Mate:119: 0005-10-008.ipt:12 ↔ 0005-10-007Suport nema.ipt:86
- Flush:64: 0005-10-008.ipt:12 ↔ 0005-10-007Suport nema.ipt:86
- Flush:65: 0005-10-009.ipt:14 ↔ 0005-10-007Suport nema.ipt:86
- Mate:120: 0005-10-1000 LM8.ipt:85 ↔ 0005-10-1018 tija 8.ipt:87
- Mate:121: 0005-10-003 Actionare seringa.ipt:41 ↔ 0005-10-1018 tija 8.ipt:87
- Flush:66: 0005-10-007Suport nema.ipt:86 ↔ 0005-10-1018 tija 8.ipt:87
- Mate:122: 0005-10-003 Actionare seringa.ipt:41 ↔ 0005-10-004 Actionare 2 seringa.ipt:42
- Mate:123: 0005-10-017 Batiu 2.ipt:50 ↔ 0005-20-1003 Switch.ipt:74
- Insert:24: 0005-10-015 suport tija.ipt:52 ↔ Surub M4 saiba piulita.iam:88
- Mate:125: 0005-10-014 Suport Bed.ipt:31 ↔ 0005-10-025 Activator senzor Y.ipt:90
- Flush:67: 0005-10-014 Suport Bed.ipt:31 ↔ 0005-10-025 Activator senzor Y.ipt:90
- Flush:68 (-5 mm): 0005-10-025 Activator senzor Y.ipt:90 ↔ 0005-10-1009 LM10uu.ipt:34
- Insert:26: 0005-10-010.ipt:15 ↔ 0005-10-1009 LM10uu.ipt:92
- Insert:27: 0005-10-010.ipt:15 ↔ 0005-10-1009 LM10uu.ipt:91
- Insert:28: 0005-10-024.ipt:83 ↔ 0005-10-1022 tiping screw.ipt:93
- Mate:126: 0005-10-024.ipt:83 ↔ 0005-10-1022 tiping screw.ipt:102
- Insert:29: 0005-10-024.ipt:84 ↔ 0005-10-1022 tiping screw.ipt:107
- Insert:30: 0005-10-024.ipt:84 ↔ 0005-10-1022 tiping screw.ipt:116
- Insert:32: 0005-10-001-Batiu.ipt:1 ↔ 0005-10-1023 ISO 4018 - M8 x 40.ipt:122
- Insert:33: 0005-10-001-Batiu.ipt:1 ↔ 0005-10-1023 ISO 4018 - M8 x 40.ipt:123
- Mate:127: 0005-10-001-Batiu.ipt:1 ↔ 0005-10-026 Suport DC in.ipt:125
- Mate:129: Inlet Module Plug Fuse Switch Male Power Socket 10A 250V 3 Pin IEC320 C14.ipt:82 ↔ 0005-10-026 Suport DC in.ipt:125
- Mate:131: 0005-10-001-Batiu.ipt:1 ↔ Inlet Module Plug Fuse Switch Male Power Socket 10A 250V 3 Pin IEC320 C14.ipt:82
- Mate:132: Inlet Module Plug Fuse Switch Male Power Socket 10A 250V 3 Pin IEC320 C14.ipt:82 ↔ 0005-10-026 Suport DC in.ipt:125
- Insert:35: ISO 4762 M3 x 16:1 ↔ ISO 7089 3:1
- Insert:36: 0005-10-011.ipt:20 ↔ ISO 4762 M3 x 16:1
- Mate:137: 0005-10-005.ipt:7 ↔ 0005-10-002 Suport1 Seringa.ipt:43
- Mate:138: 0005-10-005.ipt:7 ↔ 0005-10-002 Suport1 Seringa.ipt:43
- Flush:69: 0005-10-011.ipt:20 ↔ 0005-10-012.ipt:29
- Flush:70: 0005-10-011.ipt:20 ↔ 0005-10-012.ipt:29
- Insert:37: 0005-10-10-1003 LeadScrew 8mm x 2mmPitch.ipt:21 ↔ 0005-10-1001 NEMA17 - Motor de passo.ipt:23
- Insert:38: 0005-10-10-1003 LeadScrew 8mm x 2mmPitch.ipt:21 ↔ 0005-10-1005 ISO 1224-1 - 10 - 8 x 22 x 7.ipt:27
- Insert:39: 0005-10-006 Capac rulment.ipt:26 ↔ 0005-10-1005 ISO 1224-1 - 10 - 8 x 22 x 7.ipt:27
- Insert:40: 0005-10-011.ipt:24 ↔ Surub M3 40 mm.iam:89
- Mate:142: 0005-10-011.ipt:24 ↔ 0005-10-012.ipt:25
- Flush:71: 0005-10-011.ipt:24 ↔ 0005-10-012.ipt:29
- Flush:72: 0005-10-011.ipt:24 ↔ 0005-10-012.ipt:29
- Mate:143: 0005-10-001-Batiu.ipt:1 ↔ 00005-20-1004 PowerSupplyLedMax500.ipt:126
- Mate:144 (1 mm): 0005-10-017 Batiu 2.ipt:50 ↔ 0005-10-1001 NEMA17 - Motor de passo.ipt:58
- Mate:145 (1 mm): 0005-10-017 Batiu 2.ipt:50 ↔ 0005-10-1001 NEMA17 - Motor de passo.ipt:58
- Mate:146: 0005-10-1001 NEMA17 - Motor de passo.ipt:58 ↔ 0005-10-1010 GT2 Timing Pulley 20 Tooth.ipt:59
- Mate:147: 0005-10-001-Batiu.ipt:1 ↔ 0005-20-01 Assembly Arduino Mega RAMPS 1.4.iam:2
- Flush:73: 0005-10-001-Batiu.ipt:1 ↔ 0005-20-01 Assembly Arduino Mega RAMPS 1.4.iam:2
- Mate:148: 0005-10-017 Batiu 2.ipt:50 ↔ 00005-20-1004 PowerSupplyLedMax500.ipt:126
- Mate:149: 0005-10-024.ipt:84 ↔ 00005-20-1004 PowerSupplyLedMax500.ipt:126
- Insert:41: 0005-10-001-Batiu.ipt:1 ↔ 0005-10-1023 ISO 4018 - M8 x 40.ipt:121
- Insert:42: 0005-10-001-Batiu.ipt:1 ↔ 0005-10-1023 ISO 4018 - M8 x 40.ipt:124
- Mate:150 (120 mm): 0005-10-017 Batiu 2.ipt:50
- Mate:151: 0005-10-011.ipt:20 ↔ 0005-10-012.ipt:25
- Flush:74 (14.444 mm): 0005-10-011.ipt:20 ↔ 0005-10-021 suport senzor z.ipt:75
## Named parameters: d64_d31 = 5 mm, d217_d198 = -13 mm, d221_d205 = 1 mm, d222_d204 = 0 mm
